# Autodesk Inventor assembly: main
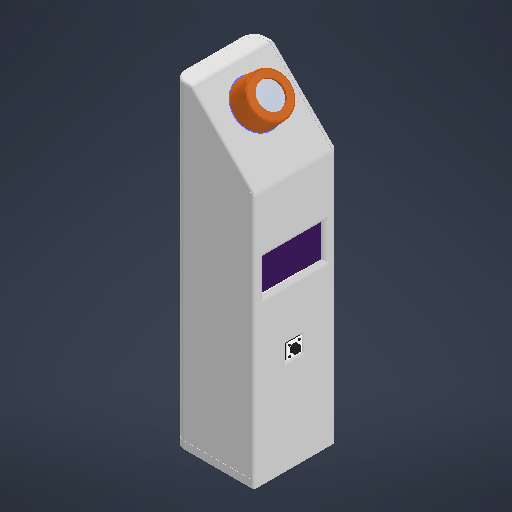
[picture p0: Inventor's stored thumbnail of the model, 512x512]
Saved by Autodesk Inventor 2027 (Build 310192060, 192F)
## iProperties
Created: 2026-07-05
Part Number: main
Document SubType Name: Assembly
Designer: User
Author: User
## Documents named in this file (6)
- G:\Github\Alkomaster\Alkomaster\Hardware\main.iam
- G:\Github\Alkomaster\Alkomaster\Hardware\Parts\Frame.ipt
- G:\Github\Alkomaster\Alkomaster\Hardware\Parts\bottom_frame.ipt
- G:\Github\Alkomaster\Alkomaster\Hardware\Parts\0.96'' OLED Display\0.96'' OLED Display.ipt
- G:\Github\Alkomaster\Alkomaster\Hardware\Parts\MQ3 Sensor\MQ3 Sensor.ipt
- G:\Github\Alkomaster\Alkomaster\Hardware\Parts\button 6x6\button 6x6.ipt
## Components (5 placed, 5 different names)
1. Frame:1 — przesuwne:1
2. bottom_frame:1 — przesuwne:1, Obrotowe:5, Obrotowe:6, Sztywne:2, Sztywne:3
3. 0.96'' OLED Display:1 — Obrotowe:5, Obrotowe:6
4. MQ3 Sensor:1 — Sztywne:3
5. button 6x6:1 — Sztywne:2
## Relationships (5: RevoluteJoint 2, WeldJoint 2, TranslationJoint 1)
- przesuwne:1 [TranslationJoint]: Frame:1 ↔ bottom_frame:1
- Obrotowe:5 [RevoluteJoint] (-2 mm): bottom_frame:1 ↔ 0.96'' OLED Display:1
- Obrotowe:6 [RevoluteJoint] (-2 mm): bottom_frame:1 ↔ 0.96'' OLED Display:1
- Sztywne:2 [WeldJoint]: bottom_frame:1 ↔ button 6x6:1
- Sztywne:3 [WeldJoint]: bottom_frame:1 ↔ MQ3 Sensor:1
